# Autodesk Inventor assembly: Screw_Joint_36T_Custom_Spacer_MIR2
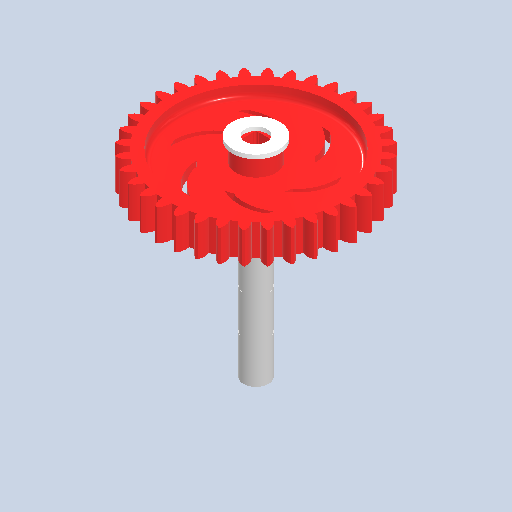
[picture p0: Inventor's stored thumbnail of the model, 512x512]
Saved by Autodesk Inventor 2025.2 (Build 292293000, 293)
## iProperties
Created: 2024-12-08
Part Number: Screw_Joint_36T_Custom_Spacer_MIR2
Document SubType Name: Assembly
Designer: joshi
Author: Aditya Koduri
## Documents named in this file (5)
- C:\Users\joshi\Desktop\3388K CAD\Screw_Joint_36T_Custom_Spacer_MIR2.iam
- C:\Users\joshi\Desktop\3388K CAD\VEX Main\Motion\Spacers\Washer Teflon\TWasher .375 OD x .03125.ipt
- C:\Users\joshi\Desktop\3388K CAD\VEX Main\Motion\Spacers\Washer Teflon.ipt
- C:\Users\joshi\Desktop\3388K CAD\VEX Main\Motion\Gears\LS 36T Gear_MIR2.ipt
- C:\Users\joshi\Desktop\3388K CAD\Thin_spacer_custom_MIR2.ipt
## Components (6 placed, 3 different names)
1. TWasher .375 OD x .03125:1 — Insert:1
2. LS 36T Gear_MIR2:1 — Insert:1, Insert:5
3. Thin_spacer_custom_MIR2:1 — Insert:2, Insert:3
4. Thin_spacer_custom_MIR2:2 — Insert:5, Insert:4
5. Thin_spacer_custom_MIR2:3 — Insert:2, Insert:4
6. Thin_spacer_custom_MIR2:4 — Insert:3
## Relationships (5: Insert 5)
- Insert:1: TWasher .375 OD x .03125:1 ↔ LS 36T Gear_MIR2:1
- Insert:5: LS 36T Gear_MIR2:1 ↔ Thin_spacer_custom_MIR2:2
- Insert:2: Thin_spacer_custom_MIR2:1 ↔ Thin_spacer_custom_MIR2:3
- Insert:4: Thin_spacer_custom_MIR2:2 ↔ Thin_spacer_custom_MIR2:3
- Insert:3: Thin_spacer_custom_MIR2:1 ↔ Thin_spacer_custom_MIR2:4
